# Autodesk Inventor assembly: Ensamblaje1
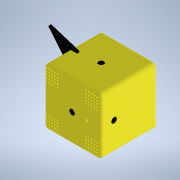
[picture p0: Inventor's stored thumbnail of the model, 180x180]
Saved by Autodesk Inventor 2021 (Build 250183000, 183)
## iProperties
Created: 2024-10-06
Part Number: Ensamblaje1
Document SubType Name: Assembly
Designer: hojan
Author: hojan
## Documents named in this file (8)
- C:\Users\hojan\Dropbox\Trabajos Personales\Nasa\assembly as cat.iam
- C:\Users\hojan\Dropbox\Trabajos Personales\Nasa\body.ipt
- C:\Users\hojan\Dropbox\Trabajos Personales\Nasa\face.ipt
- C:\Users\hojan\Dropbox\Trabajos Personales\Nasa\cat.ipt
- C:\Users\hojan\Dropbox\Trabajos Personales\Nasa\circuit.ipt
- C:\Users\hojan\Dropbox\Trabajos Personales\Nasa\sensor.ipt
- C:\Users\hojan\Dropbox\Trabajos Personales\Nasa\sensor_2.ipt
- C:\Users\hojan\Dropbox\Trabajos Personales\Nasa\screen.ipt
## Components (13 placed, 7 different names)
1. body:1 — Coincidencia:1, Coincidencia:2, Coincidencia:3, Coincidencia:4, Coincidencia:5, Coincidencia:6, Coincidencia:7, Coincidencia:8, Coincidencia:9, Coincidencia:10, Coincidencia:15, Coincidencia:16, Coincidencia:17, Coincidencia:18, Coincidencia:19, Coincidencia:20, Coincidencia:26, Coincidencia:27, Coincidencia:28
2. face:1 — Coincidencia:11, Coincidencia:12, Coincidencia:13, Coincidencia:14, Coincidencia:21, Coincidencia:22, Coincidencia:23, Coincidencia:24, Coincidencia:25, Nivelación:1, Coincidencia:26, Coincidencia:27, Coincidencia:28
3. cat:1 — Coincidencia:15, Coincidencia:16, Coincidencia:17
4. circuit:1 — Coincidencia:21, Coincidencia:22, Coincidencia:23
5. sensor:1 — Coincidencia:11, Coincidencia:12
6. sensor_2:1 — Coincidencia:1, Coincidencia:2
7. sensor_2:6 — Coincidencia:9, Coincidencia:10
8. sensor_2:8 — Coincidencia:3, Coincidencia:4
9. sensor_2:9 — Coincidencia:5, Coincidencia:6
10. sensor_2:10 — Coincidencia:7, Coincidencia:8
11. sensor:2 — Coincidencia:13, Coincidencia:14
12. cat:2 — Coincidencia:18, Coincidencia:19, Coincidencia:20
13. screen:1 — Coincidencia:24, Coincidencia:25, Nivelación:1
## Relationships (29: Mate 28, Flush 1)
- Coincidencia:1 [Mate]: body:1 ↔ sensor_2:1
- Coincidencia:2 [Mate]: body:1 ↔ sensor_2:1
- Coincidencia:3 [Mate]: body:1 ↔ sensor_2:8
- Coincidencia:4 [Mate]: body:1 ↔ sensor_2:8
- Coincidencia:5 [Mate]: body:1 ↔ sensor_2:9
- Coincidencia:6 [Mate]: body:1 ↔ sensor_2:9
- Coincidencia:7 [Mate]: body:1 ↔ sensor_2:10
- Coincidencia:8 [Mate]: body:1 ↔ sensor_2:10
- Coincidencia:9 [Mate]: body:1 ↔ sensor_2:6
- Coincidencia:10 [Mate]: body:1 ↔ sensor_2:6
- Coincidencia:11 [Mate]: face:1 ↔ sensor:1
- Coincidencia:12 [Mate]: face:1 ↔ sensor:1
- Coincidencia:13 [Mate]: face:1 ↔ sensor:2
- Coincidencia:14 [Mate]: face:1 ↔ sensor:2
- Coincidencia:15 [Mate]: body:1 ↔ cat:1
- Coincidencia:16 [Mate]: body:1 ↔ cat:1
- Coincidencia:17 [Mate]: body:1 ↔ cat:1
- Coincidencia:18 [Mate]: body:1 ↔ cat:2
- Coincidencia:19 [Mate]: body:1 ↔ cat:2
- Coincidencia:20 [Mate]: body:1 ↔ cat:2
- Coincidencia:21 [Mate]: face:1 ↔ circuit:1
- Coincidencia:22 [Mate]: face:1 ↔ circuit:1
- Coincidencia:23 [Mate]: face:1 ↔ circuit:1
- Coincidencia:24 [Mate]: face:1 ↔ screen:1
- Coincidencia:25 [Mate]: face:1 ↔ screen:1
- Nivelación:1 [Flush]: face:1 ↔ screen:1
- Coincidencia:26 [Mate]: body:1 ↔ face:1
- Coincidencia:27 [Mate]: body:1 ↔ face:1
- Coincidencia:28 [Mate]: body:1 ↔ face:1
